# Autodesk Inventor assembly: Intermediate Shaft
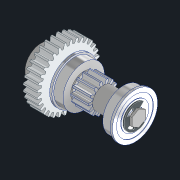
[picture p0: Inventor's stored thumbnail of the model, 180x180]
Saved by Autodesk Inventor 2022 (Build 260153000, 153)
## iProperties
Created: 2022-09-07
Part Number: Intermediate Shaft
Document SubType Name: Assembly
Designer: robpl
Author: robpl
## Documents named in this file (9)
- C:\Users\robpl\OneDrive\Documents\Inventor\2022 FRC Season\Best Coast Drive\Intermediate Shaft.iam
- C:\Users\robpl\OneDrive\Documents\Inventor\2022 FRC Season\Best Coast Drive\Intermediate Axle.ipt
- C:\Users\robpl\OneDrive\Documents\Inventor\2022 FRC Season\Best Coast Drive\14T Aluminum Spur Gear (20 DP, 3_8_ Hex Bore) (217-2699).ipt
- C:\Users\robpl\OneDrive\Documents\Inventor\2022 FRC Season\Best Coast Drive\32T Aluminum Spur Gear (20 DP, 3_8_ Hex Bore) (217-5455).ipt
- C:\Users\robpl\OneDrive\Documents\Inventor\2022 FRC Season\Best Coast Drive\22 OD 8ID 7mm Bearing.ipt
- C:\Users\robpl\OneDrive\Documents\Inventor\2022 FRC Season\Best Coast Drive\0.375 Hex ID x 1.125 OD x 0.313 WD (Flanged Bearing) (217-2735).ipt
- C:\Users\robpl\OneDrive\Documents\Inventor\2022 FRC Season\1mm 0.375in Hex Spacer.ipt
- C:\Users\robpl\OneDrive\Documents\Inventor\2022 FRC Season\Best Coast Drive\13.5mm 0.375in Hex Spacer.ipt
- C:\Users\robpl\OneDrive\Documents\Inventor\2022 FRC Season\Best Coast Drive\7mm E-Clip.ipt
## Components (10 placed, 8 different names)
1. Intermediate Axle:1 — Mate:5, Mate:6, Mate:7, Mate:8, Flush:3, Mate:9, Mate:10, Mate:11, Mate:12, Flush:4, Mate:13, Mate:14, Flush:5, Mate:20, Mate:21, Mate:22, Mate:23
2. 14T Aluminum Spur Gear (20 DP, 3_8_ Hex Bore) (217-2699):1 — Mate:5, Mate:6, Mate:17, Mate:18
3. 32T Aluminum Spur Gear (20 DP, 3_8_ Hex Bore) (217-5455):1 — Mate:7, Mate:8, Flush:3
4. 22 OD 8ID 7mm Bearing:1 — Mate:9, Mate:10
5. 0.375 Hex ID x 1.125 OD x 0.313 WD (Flanged Bearing) (217-2735):1 — Mate:11, Mate:12, Flush:4, Mate:19
6. 0.375 Hex ID x 1.125 OD x 0.313 WD (Flanged Bearing) (217-2735):2 — Mate:13, Mate:14, Flush:5, Mate:15, Mate:16
7. 1mm 0.375in Hex Spacer:1 — Mate:15, Mate:16, Mate:17
8. 13.5mm 0.375in Hex Spacer:1 — Mate:18, Mate:19
9. 7mm E-Clip:1 — Mate:20, Mate:21
10. 7mm E-Clip:2 — Mate:22, Mate:23
## Relationships (22: Mate 19, Flush 3)
- Mate:5: Intermediate Axle:1 ↔ 14T Aluminum Spur Gear (20 DP, 3_8_ Hex Bore) (217-2699):1
- Mate:6: Intermediate Axle:1 ↔ 14T Aluminum Spur Gear (20 DP, 3_8_ Hex Bore) (217-2699):1
- Mate:7: Intermediate Axle:1 ↔ 32T Aluminum Spur Gear (20 DP, 3_8_ Hex Bore) (217-5455):1
- Mate:8: Intermediate Axle:1 ↔ 32T Aluminum Spur Gear (20 DP, 3_8_ Hex Bore) (217-5455):1
- Flush:3: Intermediate Axle:1 ↔ 32T Aluminum Spur Gear (20 DP, 3_8_ Hex Bore) (217-5455):1
- Mate:9: Intermediate Axle:1 ↔ 22 OD 8ID 7mm Bearing:1
- Mate:10: Intermediate Axle:1 ↔ 22 OD 8ID 7mm Bearing:1
- Mate:11: Intermediate Axle:1 ↔ 0.375 Hex ID x 1.125 OD x 0.313 WD (Flanged Bearing) (217-2735):1
- Mate:12: Intermediate Axle:1 ↔ 0.375 Hex ID x 1.125 OD x 0.313 WD (Flanged Bearing) (217-2735):1
- Flush:4: Intermediate Axle:1 ↔ 0.375 Hex ID x 1.125 OD x 0.313 WD (Flanged Bearing) (217-2735):1
- Mate:13: Intermediate Axle:1 ↔ 0.375 Hex ID x 1.125 OD x 0.313 WD (Flanged Bearing) (217-2735):2
- Mate:14: Intermediate Axle:1 ↔ 0.375 Hex ID x 1.125 OD x 0.313 WD (Flanged Bearing) (217-2735):2
- Flush:5: Intermediate Axle:1 ↔ 0.375 Hex ID x 1.125 OD x 0.313 WD (Flanged Bearing) (217-2735):2
- Mate:15: 0.375 Hex ID x 1.125 OD x 0.313 WD (Flanged Bearing) (217-2735):2 ↔ 1mm 0.375in Hex Spacer:1
- Mate:16: 0.375 Hex ID x 1.125 OD x 0.313 WD (Flanged Bearing) (217-2735):2 ↔ 1mm 0.375in Hex Spacer:1
- Mate:17: 14T Aluminum Spur Gear (20 DP, 3_8_ Hex Bore) (217-2699):1 ↔ 1mm 0.375in Hex Spacer:1
- Mate:18: 14T Aluminum Spur Gear (20 DP, 3_8_ Hex Bore) (217-2699):1 ↔ 13.5mm 0.375in Hex Spacer:1
- Mate:19: 0.375 Hex ID x 1.125 OD x 0.313 WD (Flanged Bearing) (217-2735):1 ↔ 13.5mm 0.375in Hex Spacer:1
- Mate:20: Intermediate Axle:1 ↔ 7mm E-Clip:1
- Mate:21: Intermediate Axle:1 ↔ 7mm E-Clip:1
- Mate:22: Intermediate Axle:1 ↔ 7mm E-Clip:2
- Mate:23: Intermediate Axle:1 ↔ 7mm E-Clip:2
